# Autodesk Inventor assembly: 1.5_Bore_30in_Stroke_ROUND BODY AIR CYLINDER
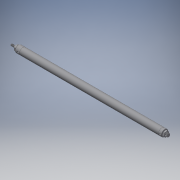
[picture p0: Inventor's stored thumbnail of the model, 180x180]
Saved by Autodesk Inventor 2018 (Build 220112000, 112)
## iProperties
Created: 2015-02-20
Part Number: 1.5_Bore_30in_Stroke_ROUND BODY AIR CYLINDER
Document SubType Name: Assembly
Designer: Administrator
Sending System: SolidWorks 2010
Major Version: 7.0
Minor Version: 0.0
Format Version: 0.0
Product Id: SolidWorks 2010
Author: Administrator
## Documents named in this file (5)
- E:\GrabCAD\Power Hawks CAD\2020 Infinite Recharge\Lift\Parts\1.5_Bore_30in_Stroke_ROUND BODY AIR CYLINDER.iam
- E:\GrabCAD\Power Hawks CAD\2020 Infinite Recharge\Lift\Parts\PistonParts\6498K507_ROUND BODY AIR CYLINDER.ipt
- E:\GrabCAD\Power Hawks CAD\2020 Infinite Recharge\Lift\Parts\PistonParts\6498K507_ROUND BODY AIR CYLINDER_2.ipt
- E:\GrabCAD\Power Hawks CAD\2020 Infinite Recharge\Lift\Parts\PistonParts\6498K507_ROUND BODY AIR CYLINDER_3.ipt
- E:\GrabCAD\Power Hawks CAD\2020 Infinite Recharge\Lift\Parts\PistonParts\6498K507_ROUND BODY AIR CYLINDER_4.ipt
## Components (4 placed, 4 different names)
1. 6498K507_ROUND BODY AIR CYLINDER_1:1 — Mate:3, Mate:4
2. 6498K507_ROUND BODY AIR CYLINDER_3:1 — Mate:1, Mate:2, Mate:3, Mate:5, Flush:1
3. 6498K507_ROUND BODY AIR CYLINDER_4:1 — Mate:1, Mate:2
4. 6498K507_ROUND BODY AIR CYLINDER_5:1 — Mate:4, Mate:5, Flush:1
## Relationships (6: Mate 5, Flush 1)
- Mate:1 (2.286 mm): 6498K507_ROUND BODY AIR CYLINDER_3:1 ↔ 6498K507_ROUND BODY AIR CYLINDER_4:1
- Mate:2: 6498K507_ROUND BODY AIR CYLINDER_3:1 ↔ 6498K507_ROUND BODY AIR CYLINDER_4:1
- Mate:3 (4.0132 mm): 6498K507_ROUND BODY AIR CYLINDER_1:1 ↔ 6498K507_ROUND BODY AIR CYLINDER_3:1
- Mate:4: 6498K507_ROUND BODY AIR CYLINDER_1:1 ↔ 6498K507_ROUND BODY AIR CYLINDER_5:1
- Mate:5: 6498K507_ROUND BODY AIR CYLINDER_3:1 ↔ 6498K507_ROUND BODY AIR CYLINDER_5:1
- Flush:1: 6498K507_ROUND BODY AIR CYLINDER_3:1 ↔ 6498K507_ROUND BODY AIR CYLINDER_5:1
